# Autodesk Inventor assembly: 220LB-ASSY_MIR
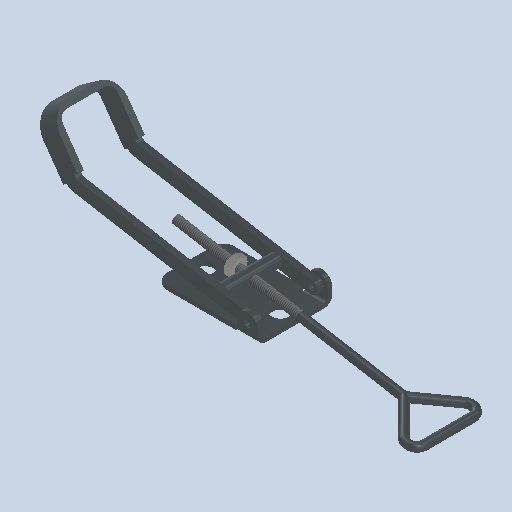
[picture p0: Inventor's stored thumbnail of the model, 512x512]
Saved by Autodesk Inventor 2025.3 (Build 293356000, 356)
## iProperties
Created: 2025-08-31
Part Number: 220LB-ASSY_MIR
Document SubType Name: Assembly
Designer: K1NG
Author: lstk1ng
## Documents named in this file (5)
- C:\Users\K1NG\Documents\PM1\DISEÑO MECANICO\220LB LOCK\220LB-ASSY_MIR.iam
- C:\Users\K1NG\Documents\PM1\DISEÑO MECANICO\220LB LOCK\BODY-220LB_MIR.ipt
- C:\Users\K1NG\Documents\PM1\DISEÑO MECANICO\220LB LOCK\GRIPPER-220LB_MIR.ipt
- C:\Users\K1NG\Documents\PM1\DISEÑO MECANICO\220LB LOCK\PLATE-220_MIR.ipt
- C:\Users\K1NG\Documents\Inventor\Content Center Files\R2025\en-US\AS 1112 (2)\AS 1112 - M2  Type 5.ipt
## Components (4 placed, 4 different names)
1. BODY-220LB_MIR:1 — Insert:1, Mate:1, Cylindrical:1
2. GRIPPER-220LB_MIR:1 — Mate:2, Cylindrical:1, Cylindrical:2
3. PLATE-220_MIR:1 — Insert:1, Mate:1
4. AS 1112 (2) - Metric M2  Type 5:1 — Mate:2, Cylindrical:2
## Relationships (5: Mate 2, CylindricalJoint 2, Insert 1)
- Insert:1: BODY-220LB_MIR:1 ↔ PLATE-220_MIR:1
- Mate:1: BODY-220LB_MIR:1 ↔ PLATE-220_MIR:1
- Mate:2: GRIPPER-220LB_MIR:1 ↔ AS 1112 (2) - Metric M2  Type 5:1
- Cylindrical:1: BODY-220LB_MIR:1 ↔ GRIPPER-220LB_MIR:1
- Cylindrical:2: GRIPPER-220LB_MIR:1 ↔ AS 1112 (2) - Metric M2  Type 5:1
